# Autodesk Inventor assembly: B-1100-1
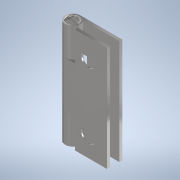
[picture p0: Inventor's stored thumbnail of the model, 180x180]
Saved by Autodesk Inventor 2022.3 (Build 263350000, 350)
## iProperties
Created: 2008-11-26
Part Number: B-1100-1
Description: STEP AP203
Document SubType Name: Assembly
Designer: Hagihara Yuya
Sending System: SolidWorks 2007
Preprocessor: SwSTEP 2.0
Title: B-1100-1.STEP
Revision Number: ANY
## Documents named in this file (4)
- C:\Users\YusukeKunita\Documents\GrabCAD\Development\BasicParts\Hinge\B-1100-1\B-1100-1.iam
- C:\Users\YusukeKunita\Documents\GrabCAD\Development\BasicParts\Hinge\B-1100-1\B-1100-1qWB__ÃÞÌ«ÙÄ.ipt
- C:\Users\YusukeKunita\Documents\GrabCAD\Development\BasicParts\Hinge\B-1100-1\B-1100-1qWA__ÃÞÌ«ÙÄ.ipt
- C:\Users\YusukeKunita\Documents\GrabCAD\Development\BasicParts\Hinge\B-1100-1\B-1100-1Vtg__ÃÞÌ«ÙÄ.ipt
## Components (3 placed, 3 different names)
1. B-1100-1qWB__ÃÞÌ«ÙÄ_1 — 回転:1
2. B-1100-1qWA__ÃÞÌ«ÙÄ_2 — 回転:1, 回転:2
3. B-1100-1Vtg__ÃÞÌ«ÙÄ_3 — 回転:2
## Relationships (2: RevoluteJoint 2)
- 回転:1 [RevoluteJoint]: B-1100-1qWB__ÃÞÌ«ÙÄ_1 ↔ B-1100-1qWA__ÃÞÌ«ÙÄ_2
- 回転:2 [RevoluteJoint]: B-1100-1qWA__ÃÞÌ«ÙÄ_2 ↔ B-1100-1Vtg__ÃÞÌ«ÙÄ_3
